# Autodesk Inventor assembly: Motor_Faulhaber_mit_Getriebe
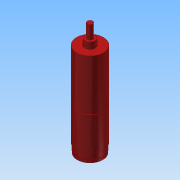
[picture p0: Inventor's stored thumbnail of the model, 180x180]
Saved by Autodesk Inventor 2015 (Build 190159000, 159)
## iProperties
Created: 2015-08-07
Part Number: Motor_Faulhaber_mit_Getriebe
Document SubType Name: Assembly
Designer: Johann
Author: Johann
## Documents named in this file (3)
- C:\Users\Johann\Documents\Uni\Bachelorarbeit\Inventor\Motor_Faulhaber_mit_Getriebe.iam
- C:\Users\Johann\Documents\Uni\Bachelorarbeit\Inventor\AM1020-(2R)-_-01\AM1020-(2R)-_-01.ipt
- C:\Users\Johann\Documents\Uni\Bachelorarbeit\Inventor\10-1\10_1 4stages.ipt
## Components (2 placed, 2 different names)
1. AM1020-(2R)-_-01:1 — Fluchtend:1, Fluchtend:2, Fluchtend:3, Passend:1, Passend:2
2. 10_1 4stages:1 — Passend:1, Passend:2, Fluchtend:4
## Relationships (6: Flush 4, Mate 2)
- Fluchtend:1 [Flush]: AM1020-(2R)-_-01:1
- Fluchtend:2 [Flush]: AM1020-(2R)-_-01:1
- Fluchtend:3 [Flush]: AM1020-(2R)-_-01:1
- Passend:1 [Mate]: AM1020-(2R)-_-01:1 ↔ 10_1 4stages:1
- Passend:2 [Mate]: AM1020-(2R)-_-01:1 ↔ 10_1 4stages:1
- Fluchtend:4 [Flush]: 10_1 4stages:1
